# Autodesk Inventor assembly: 9P Sprocket
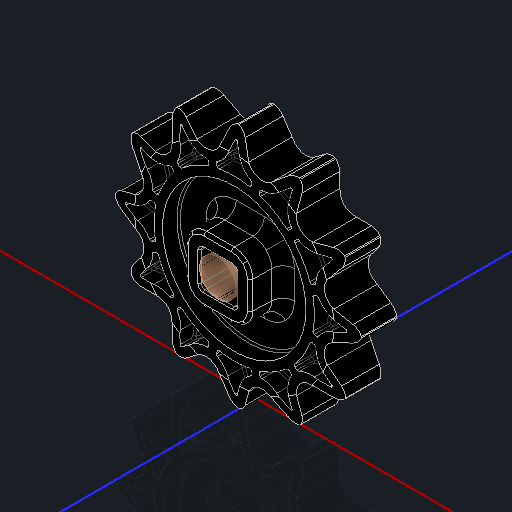
[picture p0: Inventor's stored thumbnail of the model, 512x512]
Saved by Autodesk Inventor 2025 (Build 290162000, 162)
## iProperties
Created: 2022-08-02
Part Number: 9P Sprocket
Document SubType Name: Assembly
Designer: ylu12
Author: ylu12
## Documents named in this file (3)
- D:\vex_robotics_high_stakes\hardware\cad\robpros_cad_lib\Motion\Sprockets\9P Sprocket\9P 12T Sprocket, No Insert.iam
- D:\vex_robotics_high_stakes\hardware\cad\robpros_cad_lib\Motion\Sprockets\Reference Files\9P 12T Sprocket, No Insert.ipt
- D:\vex_robotics_high_stakes\hardware\cad\robpros_cad_lib\Motion\Sprockets\9P Sprocket.iam
## Components (1 placed, 1 different names)
1. 12T — Mate:7, Mate:8, Flush:4
## Relationships (3: Mate 2, Flush 1)
- Mate:7: 12T
- Mate:8: 12T
- Flush:4: 12T
